# Autodesk Inventor assembly: 合体
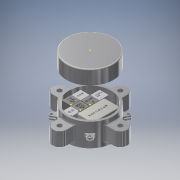
[picture p0: Inventor's stored thumbnail of the model, 180x180]
Saved by Autodesk Inventor 2018.3 (Build 223284000, 284)
## iProperties
Created: 2018-12-27
Part Number: 合体
Material: 常规
Document SubType Name: Assembly
Designer: 丁子鸣
Author: 丁子鸣
## Documents named in this file (3)
- C:\Users\丁子鸣\Desktop\比赛图\合体.iam
- C:\Users\丁子鸣\Desktop\比赛图\上部分.iam
- C:\Users\丁子鸣\Desktop\比赛图\下部分.iam
## Components (2 placed, 2 different names)
1. 上部分:1 [sub-assembly] — 配合:1, 配合:2
2. 下部分:1 [sub-assembly] — 配合:1, 配合:2
## Relationships (2: Mate 2)
- 配合:1 [Mate]: 上部分:1 ↔ 下部分:1
- 配合:2 [Mate]: 上部分:1 ↔ 下部分:1
